# Autodesk Inventor assembly: Eixo_de_movimento_001
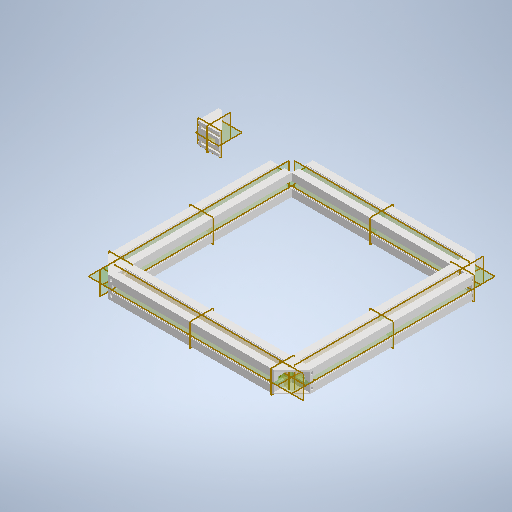
[picture p0: Inventor's stored thumbnail of the model, 512x512]
Saved by Autodesk Inventor 2025.2 (Build 292293000, 293)
## iProperties
Created: 2025-04-08
Part Number: Eixo_de_movimento_001
Document SubType Name: Assembly
Designer: ishad
Author: ishad
## Documents named in this file (3)
- C:\Users\ishad\Documents\Inventor\Eixo_de_movimento_linear\Eixo_de_movimento_001.iam
- C:\Users\ishad\Documents\Inventor\Sessao_6_28_03_2025\Perfil 20_500.ipt
- C:\Users\ishad\Downloads\Soporte_2020_0001.ipt
## Components (8 placed, 2 different names)
1. Perfil 20_500:1 — Mate:1, Mate:2, Mate:5, Flush:1, Flush:2, Symmetry:1
2. Perfil 20_500:2 — Mate:3, Mate:4, Mate:9, Flush:5, Angle:1, Mate:10, Mate:11, Symmetry:1, Mate:12, Flush:6, Flush:7
3. Perfil 20_500:3 — Flush:8, Mate:13, Flush:9, Mate:14
4. Perfil 20_500:5 — Mate:6, Flush:3, Mate:7, Mate:8, Flush:4
5. Soporte_2020_0001:1 — Mate:5, Flush:1, Flush:2, Mate:6, Flush:3, Mate:7
6. Soporte_2020_0001:2 — Mate:8, Flush:4, Mate:9, Flush:5, Angle:1, Mate:10, Mate:11
7. Soporte_2020_0001:3 — Mate:12, Flush:6, Flush:7, Flush:8, Mate:13, Flush:9, Mate:14
8. Soporte_2020_0001:4
## Relationships (25: Mate 14, Flush 9, Angle 1, Symmetry 1)
- Mate:1: Perfil 20_500:1
- Mate:2: Perfil 20_500:1
- Mate:3: Perfil 20_500:2
- Mate:4: Perfil 20_500:2
- Mate:5: Perfil 20_500:1 ↔ Soporte_2020_0001:1
- Flush:1: Perfil 20_500:1 ↔ Soporte_2020_0001:1
- Flush:2: Perfil 20_500:1 ↔ Soporte_2020_0001:1
- Mate:6: Perfil 20_500:5 ↔ Soporte_2020_0001:1
- Flush:3: Perfil 20_500:5 ↔ Soporte_2020_0001:1
- Mate:7 (1.4 mm): Perfil 20_500:5 ↔ Soporte_2020_0001:1
- Mate:8: Perfil 20_500:5 ↔ Soporte_2020_0001:2
- Flush:4: Perfil 20_500:5 ↔ Soporte_2020_0001:2
- Mate:9: Perfil 20_500:2 ↔ Soporte_2020_0001:2
- Flush:5: Perfil 20_500:2 ↔ Soporte_2020_0001:2
- Angle:1 (90 deg): Perfil 20_500:2 ↔ Soporte_2020_0001:2
- Mate:10: Perfil 20_500:2 ↔ Soporte_2020_0001:2
- Mate:11 (-85 mm): Perfil 20_500:2 ↔ Soporte_2020_0001:2
- Symmetry:1: Perfil 20_500:1 ↔ Perfil 20_500:2
- Mate:12: Perfil 20_500:2 ↔ Soporte_2020_0001:3
- Flush:6: Perfil 20_500:2 ↔ Soporte_2020_0001:3
- Flush:7: Perfil 20_500:2 ↔ Soporte_2020_0001:3
- Flush:8: Perfil 20_500:3 ↔ Soporte_2020_0001:3
- Mate:13: Perfil 20_500:3 ↔ Soporte_2020_0001:3
- Flush:9: Perfil 20_500:3 ↔ Soporte_2020_0001:3
- Mate:14: Perfil 20_500:3 ↔ Soporte_2020_0001:3
